# Autodesk Inventor assembly: servo motor power HD1501MG
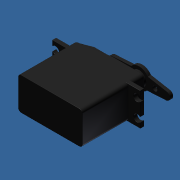
[picture p0: Inventor's stored thumbnail of the model, 180x180]
Saved by Autodesk Inventor 2014 (Build 180170000, 170)
## iProperties
Created: 2010-09-11
Part Number: servo motor power HD1501MG
Document SubType Name: Assembly
Designer: LEFO
Author: LEFO
## Documents named in this file (4)
- C:\Users\Lefo\Documents\Inventor\academy\servo power HD1501MG\servo motor power HD1501MG.iam
- C:\Users\Lefo\Documents\Inventor\academy\servo power HD1501MG\carcaza servo power HD1501MG.ipt
- C:\Users\Lefo\Documents\Inventor\academy\servo power HD1501MG\pinhon servo.ipt
- C:\Users\Lefo\Documents\Inventor\academy\servo power HD1501MG\acople estrella2 servo.ipt
## Components (3 placed, 3 different names)
1. carcaza servo power HD1501MG:1 — Insert:1
2. pinhon servo:1 — Insert:1, Insert:2
3. acople estrella2 servo:1 — Insert:2
## Relationships (2: Insert 2)
- Insert:1 (0.5 mm): carcaza servo power HD1501MG:1 ↔ pinhon servo:1
- Insert:2 (0.3 mm): pinhon servo:1 ↔ acople estrella2 servo:1
